# Autodesk Inventor assembly: StraightMF134
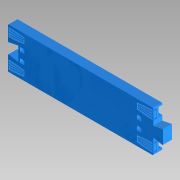
[picture p0: Inventor's stored thumbnail of the model, 180x180]
Saved by Autodesk Inventor 2021 (Build 250183000, 183)
## iProperties
Created: 2021-03-01
Part Number: StraightMF134
Document SubType Name: Assembly
Designer: kumagai
Author: kumagai
## Documents named in this file (5)
- X:\Develop\CAD\PlaRails\StraightRail\StraightRail_i\StraightMF134.iam
- X:\Develop\CAD\PlaRails\RailJointMale.ipt
- X:\Develop\CAD\PlaRails\RailJointFemale.ipt
- X:\Develop\CAD\PlaRails\GlobalParameter.ipt
- X:\Develop\CAD\PlaRails\StraightRail\StraightRail_i.iam
## Components (2 placed, 2 different names)
1. M1 — フラッシュ:1, フラッシュ:3, フラッシュ:4
2. F2 — フラッシュ:6, フラッシュ:7, フラッシュ:8
## Relationships (6: Flush 6)
- フラッシュ:1 [Flush]: M1
- フラッシュ:3 [Flush] (-52.25 mm): M1
- フラッシュ:4 [Flush]: M1
- フラッシュ:6 [Flush]: F2
- フラッシュ:7 [Flush] (-52.25 mm): F2
- フラッシュ:8 [Flush]: F2
## Named parameters: Length = 134.5 mm, ConnectorLength = 15 mm, Offset = 52.25 mm
